# Autodesk Inventor assembly: ChessBoardOld
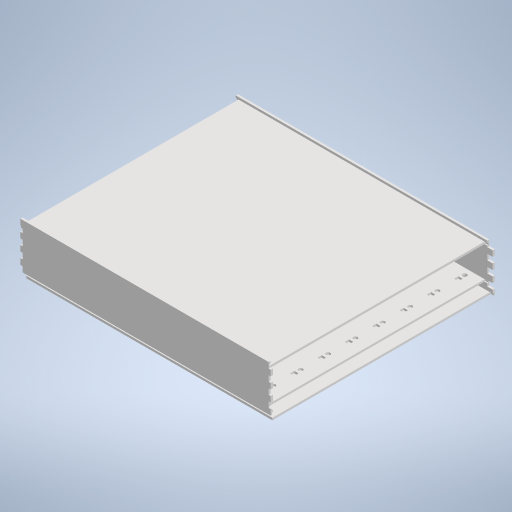
[picture p0: Inventor's stored thumbnail of the model, 512x512]
Saved by Autodesk Inventor 2024.3 (Build 283343010, 343A)
## iProperties
Created: 2025-04-25
Part Number: ChessBoardOld
Document SubType Name: Assembly
Designer: powellee
Author: powellee
## iProperties of the stored document Floor.ipt
Created: 2025-04-23
Part Number: Floor
Material: Generic
Document SubType Name: Modeling
Designer: powel
Density: 1 g/cm^3
Appearance: Default
Author: powel
Sending System: Autodesk Inventor 2025
## iProperties of the stored document Side Wall.ipt
Created: 2025-04-21
Part Number: Side Wall
Material: Generic
Document SubType Name: Modeling
Designer: powel
Density: 1 g/cm^3
Appearance: Default
Author: powel
Sending System: Autodesk Inventor 2025
## iProperties of the stored document ChessBoard.iam
Created: 2025-04-21
Part Number: ChessBoard
Document SubType Name: Assembly
Designer: powel
Author: powel
Sending System: Autodesk Inventor 2025
## iProperties of the stored document LED Holder.ipt
Created: 2025-04-21
Part Number: LED Holder
Material: Generic
Document SubType Name: Modeling
Designer: powel
Density: 1 g/cm^3
Appearance: Default
Author: powel
Sending System: Autodesk Inventor 2025
## iProperties of the stored document Side Wall_MIR.ipt
Created: 2025-04-21
Part Number: Side Wall_MIR
Material: Generic
Document SubType Name: Modeling
Designer: powel
Density: 1 g/cm^3
Appearance: Default
Author: powel
Sending System: Autodesk Inventor 2025
## Documents named in this file (11)
- **D:\School\Chess Set\ChessBoardOld.iam*LocalDocs*xAaaaaicaAaaaaaaaAaaaa4hnUa*Floor.ipt
- **D:\School\Chess Set\ChessBoardOld.iam*LocalDocs*xAaaaahaaAaaaaaaaAaaaq3np5f*Side Wall.ipt
- **D:\School\Chess Set\ChessBoardOld.iam*LocalDocs*xAaaaqkaaAaaaaaaaAaaaa1msYa*ChessBoard.iam
- **D:\School\Chess Set\ChessBoardOld.iam*LocalDocs*xAaaaq4daAaaaaaaaAaaaafnuXa*LED Holder.ipt
- **D:\School\Chess Set\ChessBoardOld.iam*LocalDocs*xAaaaqycaAaaaaaaaAaaaah4jQf*Side Wall_MIR.ipt
- D:\School\Chess Set\ChessBoardOld.iam
- D:\School\Chess Set\ChessBoard.iam
- D:\School\Chess Set\Floor.ipt
- D:\School\Chess Set\LED Holder.ipt
- D:\School\Chess Set\Side Wall.ipt
- D:\School\Chess Set\Side Wall_MIR.ipt
## Components (1 placed, 1 different names)
1. ChessBoard:1 [sub-assembly]
## Named parameters: Finish1_Area = 700.976, Finish2_Area = 737.28
note: some values were not read from the file. Shown as the stored number, unit unknown: "Finish1_Area", "Finish2_Area".
